# Autodesk Inventor assembly: extruder
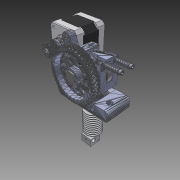
[picture p0: Inventor's stored thumbnail of the model, 180x180]
Saved by Autodesk Inventor 2014 (Build 180170000, 170)
## iProperties
Created: 2014-01-11
Part Number: extruder
Document SubType Name: Assembly
Designer: buben
Mass: 277.166 g
Surface Area: 918.506 cm^2
Volume: 186.817 cm^3
Density: 1.48362 g/cm^3
Author: buben
## Documents named in this file (20)
- C:\Users\buben\Documents\GitHub\bacon\inventor files\assemblies\extruder.iam
- C:\Users\buben\Documents\GitHub\bacon\inventor files\3rd party components\nema_17_stepper\Imported Components\NEMA 17\NEMA 17.iam
- C:\Users\buben\Documents\GitHub\bacon\inventor files\utils\washer_m3.ipt
- C:\Users\buben\Documents\Inventor\Content Center Files\R2014\en-US\ISO 4762(2)\ISO 4762 - M3 x 10ISO.ipt
- C:\Users\buben\Documents\GitHub\bacon\inventor files\3rd party components\bearing_608\Imported Components\608RS\608RS.ipt
- C:\Users\buben\Documents\Inventor\Content Center Files\R2014\en-US\ANSI B18.3.1M(6)\ANSI B18.3.1M - M3x0,5 x 35(1).ipt
- C:\Users\buben\Documents\GitHub\bacon\inventor files\utils\extruder_bearing_shaft.ipt
- C:\Users\buben\Documents\GitHub\bacon\inventor files\utils\washer_m8.ipt
- C:\Users\buben\Documents\Inventor\Content Center Files\R2014\en-US\CSN EN 24032\ISO 4032 - M8CSN EN.ipt
- C:\Users\buben\Documents\Inventor\Content Center Files\R2014\en-US\CSN EN 24014\ISO 4014 - M8 x 55CSN EN.ipt
- C:\Users\buben\Documents\Inventor\Content Center Files\R2014\en-US\ISO 7040\ISO 7040 - M3.ipt
- C:\Users\buben\Documents\GitHub\bacon\inventor files\assemblies\extruder\Design Accelerator\Compress Spring2.iam
- C:\Users\buben\Documents\Inventor\Content Center Files\R2014\en-US\ANSI B18.3.1M(6)\ANSI B18.3.1M - M3x0,5 x 60(1).ipt
- C:\Users\buben\Documents\GitHub\bacon\inventor files\utils\ds_hotend\hotend.iam
- C:\Users\buben\Documents\GitHub\bacon\inventor files\3rd party components\gregs wade\block.ipt
- C:\Users\buben\Documents\GitHub\bacon\inventor files\3rd party components\gregs wade\iddler.ipt
- C:\Users\buben\Documents\GitHub\bacon\inventor files\3rd party components\gregs wade\big_gear.ipt
- C:\Users\buben\Documents\GitHub\bacon\inventor files\3rd party components\gregs wade\small_gear.ipt
- C:\Users\buben\Documents\Inventor\Content Center Files\R2014\en-US\ISO 4762(2)\ISO 4762 - M3 x 8ISO.ipt
- C:\Users\buben\Documents\Inventor\Content Center Files\R2014\en-US\CSN EN 24032\ISO 4032 - M3CSN EN.ipt
## Components (37 placed, 19 different names)
1. NEMA 17:1 [sub-assembly] — Mate:8, Mate:9, Mate:47, Mate:48, Tangent:17, Tangent:18, Tangent:19, Mate:73
2. CSN 02 1702 B B 3,2:1 — Insert:2, Mate:63
3. CSN 02 1702 B B 3,2:2 — Insert:1, Mate:61
4. CSN 02 1702 B B 3,2:3 — Insert:3, Mate:62
5. ISO 4762 M3 x 10:1 — Insert:1, Mate:48, Tangent:10
6. ISO 4762 M3 x 10:2 — Insert:2, Mate:9, Tangent:9
7. ISO 4762 M3 x 10:3 — Insert:3, Mate:8
8. 608RS:1 — Mate:25, Mate:26, Tangent:5, Tangent:6, Mate:55
9. 608RS:2 — Mate:27, Tangent:3, Tangent:4, Mate:54
10. Forged Socket Head Cap Screw - Metric M3x0,5 x 35:1 — Insert:4, Mate:34, Mate:36, Tangent:1, Tangent:2, Tangent:7, Tangent:8
11. CSN 02 1702 B B 3,2:4 — Insert:4, Mate:56
12. CSN 02 1702 B B 3,2:5 — Mate:34, Mate:35, Mate:58
13. extruder_bearing_shaft:1 — Mate:14, Tangent:13, Tangent:14, Mate:65
14. 608RS:3 — Mate:14, Mate:66
15. CSN 02 1702 B B 8,4:1 — Mate:17, Mate:18, Mate:19, Mate:20
16. CSN 02 1702 B B 8,4:2 — Mate:19, Mate:20, Mate:23, Mate:25
17. CSN 02 1702 B B 8,4:3 — Mate:17, Mate:18, Mate:68
18. CSN 02 1702 B B 8,4:4 — Mate:27, Mate:28, Mate:32
19. CSN EN 24014 M8 x 55:1 — Mate:23, Mate:26, Mate:28, Mate:31, Tangent:15, Tangent:16, Angle:3, Mate:67
20. CSN EN 24032 M8:1 — Mate:29, Mate:30, Flush:2
21. CSN EN 24032 M8:2 — Mate:29, Mate:30, Flush:2, Mate:31, Mate:32
22. DIN EN ISO 7040 M3:1 — Mate:35, Mate:36
23. CSN 02 1702 B B 3,2:6 — Mate:41, Mate:42, Mate:44, Mate:60
24. CSN 02 1702 B B 3,2:7 — Mate:40, Flush:3, Mate:46, Mate:59
25. Compress Spring:1 [sub-assembly] — Mate:40, Flush:3, Mate:45
26. Compress Spring:2 [sub-assembly] — Mate:41, Mate:42, Mate:43
27. CSN 02 1702 B B 3,2:8 — Mate:45, Mate:46, Insert:6
28. CSN 02 1702 B B 3,2:9 — Mate:43, Mate:44, Insert:5
29. Forged Socket Head Cap Screw - Metric M3x0,5 x 60:1 — Insert:6
30. Forged Socket Head Cap Screw - Metric M3x0,5 x 60:2 — Insert:5
31. hotend:1 [sub-assembly] — Mate:64, Tangent:11, Tangent:12, Angle:2
32. block:1 — Mate:47, Mate:52, Mate:53, Flush:4, Tangent:1, Tangent:2, Tangent:3, Tangent:4, Mate:54, Tangent:5, Tangent:6, Mate:55, Mate:57, Angle:1, Tangent:9, Tangent:10, Mate:61, Mate:62, Mate:63, Mate:64, Tangent:11, Tangent:12, Angle:2
33. iddler:1 — Tangent:7, Tangent:8, Mate:56, Mate:57, Mate:58, Mate:59, Mate:60, Angle:1, Tangent:13, Tangent:14, Mate:65, Mate:66
34. big_gear:1 — Tangent:15, Tangent:16, Angle:3, Mate:67, Mate:68
35. small_gear:1 — Mate:69, Mate:71, Mate:72, Tangent:18, Tangent:19, Mate:73
36. ISO 4762 M3 x 8:1 — Mate:70, Tangent:17
37. CSN EN 24032 M3:1 — Mate:69, Mate:70, Mate:71, Mate:72
## Relationships (81: Mate 50, Tangent 19, Insert 6, Flush 3, Angle 3)
- Insert:1: CSN 02 1702 B B 3,2:2 ↔ ISO 4762 M3 x 10:1
- Insert:2: CSN 02 1702 B B 3,2:1 ↔ ISO 4762 M3 x 10:2
- Insert:3: CSN 02 1702 B B 3,2:3 ↔ ISO 4762 M3 x 10:3
- Mate:8: NEMA 17:1 ↔ ISO 4762 M3 x 10:3
- Mate:9: NEMA 17:1 ↔ ISO 4762 M3 x 10:2
- Insert:4: Forged Socket Head Cap Screw - Metric M3x0,5 x 35:1 ↔ CSN 02 1702 B B 3,2:4
- Mate:14: extruder_bearing_shaft:1 ↔ 608RS:3
- Mate:17: CSN 02 1702 B B 8,4:1 ↔ CSN 02 1702 B B 8,4:3
- Mate:18: CSN 02 1702 B B 8,4:1 ↔ CSN 02 1702 B B 8,4:3
- Mate:19: CSN 02 1702 B B 8,4:1 ↔ CSN 02 1702 B B 8,4:2
- Mate:20: CSN 02 1702 B B 8,4:1 ↔ CSN 02 1702 B B 8,4:2
- Mate:23: CSN 02 1702 B B 8,4:2 ↔ CSN EN 24014 M8 x 55:1
- Mate:25: 608RS:1 ↔ CSN 02 1702 B B 8,4:2
- Mate:26: 608RS:1 ↔ CSN EN 24014 M8 x 55:1
- Mate:27: 608RS:2 ↔ CSN 02 1702 B B 8,4:4
- Mate:28: CSN 02 1702 B B 8,4:4 ↔ CSN EN 24014 M8 x 55:1
- Mate:29: CSN EN 24032 M8:1 ↔ CSN EN 24032 M8:2
- Mate:30: CSN EN 24032 M8:1 ↔ CSN EN 24032 M8:2
- Flush:2: CSN EN 24032 M8:1 ↔ CSN EN 24032 M8:2
- Mate:31: CSN EN 24014 M8 x 55:1 ↔ CSN EN 24032 M8:2
- Mate:32: CSN 02 1702 B B 8,4:4 ↔ CSN EN 24032 M8:2
- Mate:34: Forged Socket Head Cap Screw - Metric M3x0,5 x 35:1 ↔ CSN 02 1702 B B 3,2:5
- Mate:35: CSN 02 1702 B B 3,2:5 ↔ DIN EN ISO 7040 M3:1
- Mate:36: Forged Socket Head Cap Screw - Metric M3x0,5 x 35:1 ↔ DIN EN ISO 7040 M3:1
- Mate:40: CSN 02 1702 B B 3,2:7 ↔ Compress Spring:1
- Flush:3: CSN 02 1702 B B 3,2:7 ↔ Compress Spring:1
- Mate:41: CSN 02 1702 B B 3,2:6 ↔ Compress Spring:2
- Mate:42: CSN 02 1702 B B 3,2:6 ↔ Compress Spring:2
- Mate:43: Compress Spring:2 ↔ CSN 02 1702 B B 3,2:9
- Mate:44: CSN 02 1702 B B 3,2:6 ↔ CSN 02 1702 B B 3,2:9
- Mate:45: Compress Spring:1 ↔ CSN 02 1702 B B 3,2:8
- Mate:46: CSN 02 1702 B B 3,2:7 ↔ CSN 02 1702 B B 3,2:8
- Insert:5: CSN 02 1702 B B 3,2:9 ↔ Forged Socket Head Cap Screw - Metric M3x0,5 x 60:2
- Insert:6: CSN 02 1702 B B 3,2:8 ↔ Forged Socket Head Cap Screw - Metric M3x0,5 x 60:1
- Mate:47: NEMA 17:1 ↔ block:1
- Mate:48: NEMA 17:1 ↔ ISO 4762 M3 x 10:1
- Mate:52: block:1
- Mate:53: block:1
- Flush:4: block:1
- Tangent:1 (0.2 mm): Forged Socket Head Cap Screw - Metric M3x0,5 x 35:1 ↔ block:1
- Tangent:2 (0.2 mm): Forged Socket Head Cap Screw - Metric M3x0,5 x 35:1 ↔ block:1
- Tangent:3: 608RS:2 ↔ block:1
- Tangent:4: 608RS:2 ↔ block:1
- Mate:54: 608RS:2 ↔ block:1
- Tangent:5: 608RS:1 ↔ block:1
- Tangent:6: 608RS:1 ↔ block:1
- Mate:55 (1 mm): 608RS:1 ↔ block:1
- Tangent:7: Forged Socket Head Cap Screw - Metric M3x0,5 x 35:1 ↔ iddler:1
- Tangent:8: Forged Socket Head Cap Screw - Metric M3x0,5 x 35:1 ↔ iddler:1
- Mate:56: CSN 02 1702 B B 3,2:4 ↔ iddler:1
- Mate:57 (0.4 mm): block:1 ↔ iddler:1
- Mate:58: CSN 02 1702 B B 3,2:5 ↔ iddler:1
- Mate:59: CSN 02 1702 B B 3,2:7 ↔ iddler:1
- Mate:60: CSN 02 1702 B B 3,2:6 ↔ iddler:1
- Angle:1 (0 deg): block:1 ↔ iddler:1
- Tangent:9 (0.2 mm): ISO 4762 M3 x 10:2 ↔ block:1
- Tangent:10 (0.6 mm): ISO 4762 M3 x 10:1 ↔ block:1
- Mate:61: CSN 02 1702 B B 3,2:2 ↔ block:1
- Mate:62: CSN 02 1702 B B 3,2:3 ↔ block:1
- Mate:63: CSN 02 1702 B B 3,2:1 ↔ block:1
- Mate:64 (1 mm): hotend:1 ↔ block:1
- Tangent:11: hotend:1 ↔ block:1
- Tangent:12: hotend:1 ↔ block:1
- Angle:2 (0 deg): hotend:1 ↔ block:1
- Tangent:13: extruder_bearing_shaft:1 ↔ iddler:1
- Tangent:14: extruder_bearing_shaft:1 ↔ iddler:1
- Mate:65: extruder_bearing_shaft:1 ↔ iddler:1
- Mate:66: 608RS:3 ↔ iddler:1
- Tangent:15 (0.005 mm): CSN EN 24014 M8 x 55:1 ↔ big_gear:1
- Tangent:16 (0.005 mm): CSN EN 24014 M8 x 55:1 ↔ big_gear:1
- Angle:3 (180 deg): CSN EN 24014 M8 x 55:1 ↔ big_gear:1
- Mate:67: CSN EN 24014 M8 x 55:1 ↔ big_gear:1
- Mate:68: CSN 02 1702 B B 8,4:3 ↔ big_gear:1
- Mate:69 (0.2 mm): small_gear:1 ↔ CSN EN 24032 M3:1
- Mate:70: ISO 4762 M3 x 8:1 ↔ CSN EN 24032 M3:1
- Mate:71: small_gear:1 ↔ CSN EN 24032 M3:1
- Mate:72 (0.2 mm): small_gear:1 ↔ CSN EN 24032 M3:1
- Tangent:17: NEMA 17:1 ↔ ISO 4762 M3 x 8:1
- Tangent:18 (0.2 mm): NEMA 17:1 ↔ small_gear:1
- Tangent:19 (0.2 mm): NEMA 17:1 ↔ small_gear:1
- Mate:73 (0.8 mm): NEMA 17:1 ↔ small_gear:1
